# Autodesk Inventor assembly: assemble
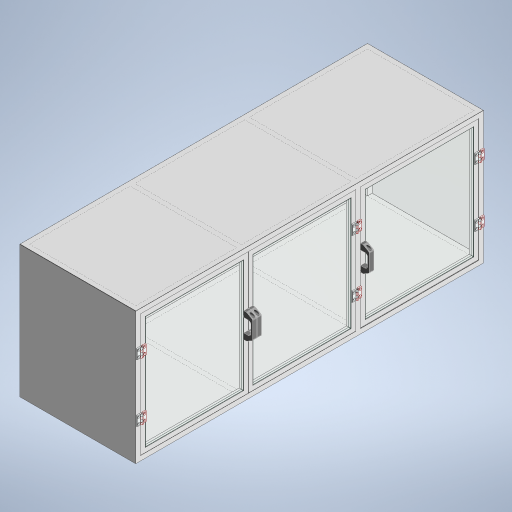
[picture p0: Inventor's stored thumbnail of the model, 512x512]
Saved by Autodesk Inventor 2023.5 (Build 275446000, 446)
## iProperties
Created: 2025-04-17
Part Number: assemble
Document SubType Name: Assembly
Designer: LENOVO
Author: LENOVO
## Documents named in this file (9)
- E:\filedata\invertorfile\tudien\assemble.iam
- E:\filedata\invertorfile\tudien\tudien2.ipt
- E:\filedata\invertorfile\tudien\door1_cover.iam
- E:\filedata\invertorfile\tudien\door2_cover.iam
- E:\filedata\invertorfile\tudien\Industrial Hinge 40 x 40\Industrial Hinge 40 x 40.ipt
- E:\filedata\invertorfile\tudien\cover1.ipt
- E:\filedata\invertorfile\tudien\cover2.ipt
- E:\filedata\invertorfile\tudien\cover3.ipt
- E:\filedata\invertorfile\tudien\cover4.ipt
## Components (15 placed, 8 different names)
1. tudien2:1 — Mate:7, Flush:4, Mate:8, Flush:5, Mate:9, Mate:10, Mate:11, Mate:12, Flush:6, Flush:7, Flush:8, Flush:9, Mate:13, Flush:10, Mate:15, Mate:16, Mate:17, Flush:11, Mate:18, Mate:19, Mate:20
2. door2_cover:1 [sub-assembly] — Mate:21, Flush:15, Mate:22
3. Industrial Hinge 40 x 40:1 — Mate:7, Flush:4, Flush:14, Mate:20, Flush:17, Mate:26
4. Industrial Hinge 40 x 40:2 — Mate:8, Flush:5, Flush:14, Mate:25
5. Industrial Hinge 40 x 40:3 — Mate:9, Mate:17, Flush:13, Mate:23
6. Industrial Hinge 40 x 40:5 — Mate:10, Flush:11, Flush:13, Mate:19, Flush:16, Mate:24
7. Industrial Hinge 40 x 40:6 — Mate:11, Mate:15, Flush:12, Mate:21
8. Industrial Hinge 40 x 40:7 — Mate:12, Mate:16, Flush:12, Mate:18, Flush:15, Mate:22
9. cover1:1 — Flush:6, Mate:14
10. cover2:1 — Flush:7
11. cover3:1 — Flush:8
12. cover4:1 — Flush:9
13. cover4:2 — Mate:13, Flush:10, Mate:14
14. door2_cover:2 [sub-assembly] — Mate:23, Flush:16, Mate:24
15. door1_cover:1 [sub-assembly] — Mate:25, Flush:17, Mate:26
## Relationships (34: Mate 20, Flush 14)
- Mate:7: tudien2:1 ↔ Industrial Hinge 40 x 40:1
- Flush:4: tudien2:1 ↔ Industrial Hinge 40 x 40:1
- Mate:8: tudien2:1 ↔ Industrial Hinge 40 x 40:2
- Flush:5: tudien2:1 ↔ Industrial Hinge 40 x 40:2
- Mate:9: tudien2:1 ↔ Industrial Hinge 40 x 40:3
- Mate:10: tudien2:1 ↔ Industrial Hinge 40 x 40:5
- Mate:11: tudien2:1 ↔ Industrial Hinge 40 x 40:6
- Mate:12: tudien2:1 ↔ Industrial Hinge 40 x 40:7
- Flush:6: tudien2:1 ↔ cover1:1
- Flush:7: tudien2:1 ↔ cover2:1
- Flush:8: tudien2:1 ↔ cover3:1
- Flush:9: tudien2:1 ↔ cover4:1
- Mate:13: tudien2:1 ↔ cover4:2
- Flush:10: tudien2:1 ↔ cover4:2
- Mate:14: cover1:1 ↔ cover4:2
- Mate:15 (-20 mm): tudien2:1 ↔ Industrial Hinge 40 x 40:6
- Mate:16 (-20 mm): tudien2:1 ↔ Industrial Hinge 40 x 40:7
- Mate:17 (-20 mm): tudien2:1 ↔ Industrial Hinge 40 x 40:3
- Flush:11: tudien2:1 ↔ Industrial Hinge 40 x 40:5
- Flush:12 (250 mm): Industrial Hinge 40 x 40:6 ↔ Industrial Hinge 40 x 40:7
- Flush:13 (250 mm): Industrial Hinge 40 x 40:3 ↔ Industrial Hinge 40 x 40:5
- Flush:14 (250 mm): Industrial Hinge 40 x 40:1 ↔ Industrial Hinge 40 x 40:2
- Mate:18 (120 mm): tudien2:1 ↔ Industrial Hinge 40 x 40:7
- Mate:19 (120 mm): tudien2:1 ↔ Industrial Hinge 40 x 40:5
- Mate:20 (120 mm): tudien2:1 ↔ Industrial Hinge 40 x 40:1
- Mate:21: door2_cover:1 ↔ Industrial Hinge 40 x 40:6
- Flush:15 (120 mm): door2_cover:1 ↔ Industrial Hinge 40 x 40:7
- Mate:22 (-20 mm): door2_cover:1 ↔ Industrial Hinge 40 x 40:7
- Mate:23: Industrial Hinge 40 x 40:3 ↔ door2_cover:2
- Flush:16 (120 mm): Industrial Hinge 40 x 40:5 ↔ door2_cover:2
- Mate:24 (-20 mm): Industrial Hinge 40 x 40:5 ↔ door2_cover:2
- Mate:25: Industrial Hinge 40 x 40:2 ↔ door1_cover:1
- Flush:17 (120 mm): Industrial Hinge 40 x 40:1 ↔ door1_cover:1
- Mate:26 (-20 mm): Industrial Hinge 40 x 40:1 ↔ door1_cover:1
